# Autodesk Inventor assembly: AXp2+p
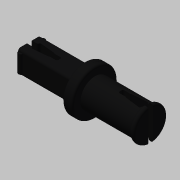
[picture p0: Inventor's stored thumbnail of the model, 180x180]
Saved by Autodesk Inventor 2019.3 (Build 233278000, 278)
## iProperties
Created: 2019-02-08
Part Number: AXp2+p
Document SubType Name: Assembly
Designer: Varga Daniel
Author: Varga Daniel
## Documents named in this file (4)
- C:\!_Dani\!_cloud\OneDrive\!_munka\Revolution\RevvyDemoKit\Structural parts\Axles\AXp2p.iam
- C:\!_Dani\!_cloud\OneDrive\!_munka\Revolution\RevvyDemoKit\Structural parts\Connetor Pins\Connector_pin_collar.ipt
- C:\!_Dani\!_cloud\OneDrive\!_munka\Revolution\RevvyDemoKit\Structural parts\Connetor Pins\Connector_pin_stick.ipt
- C:\!_Dani\!_cloud\OneDrive\!_munka\Revolution\RevvyDemoKit\Structural parts\Connetor Pins\Connector_pin_stick_square.ipt
## Components (4 placed, 3 different names)
1. Connector_pin_stick:1 — Mate:1, Mate:2, Angle:1
2. Connector_pin_stick_square:1 — Mate:5, Mate:6, Angle:1, Angle:2, Tangent:1, Angle:3, Tangent:2
3. Connector_pin_collar:1 — Mate:1, Mate:2, Mate:3, Mate:4
4. Connector_pin_collar:2 — Mate:3, Mate:4, Mate:5, Mate:6
## Relationships (11: Mate 6, Angle 3, Tangent 2)
- Mate:1: Connector_pin_stick:1 ↔ Connector_pin_collar:1
- Mate:2: Connector_pin_stick:1 ↔ Connector_pin_collar:1
- Mate:3: Connector_pin_collar:1 ↔ Connector_pin_collar:2
- Mate:4: Connector_pin_collar:1 ↔ Connector_pin_collar:2
- Mate:5: Connector_pin_stick_square:1 ↔ Connector_pin_collar:2
- Mate:6: Connector_pin_stick_square:1 ↔ Connector_pin_collar:2
- Angle:1 (0 deg): Connector_pin_stick:1 ↔ Connector_pin_stick_square:1
- Angle:2 (0 deg): Connector_pin_stick_square:1
- Tangent:1: Connector_pin_stick_square:1
- Angle:3 (0 deg): Connector_pin_stick_square:1
- Tangent:2: Connector_pin_stick_square:1
